# Autodesk Inventor assembly: NINA-W102 Module
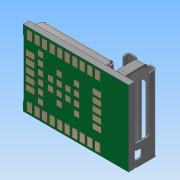
[picture p0: Inventor's stored thumbnail of the model, 180x180]
Saved by Autodesk Inventor 2016 (Build 200138000, 138)
## iProperties
Created: 2019-08-17
Part Number: NINA-W102 Module
Document SubType Name: Assembly
Designer: Orest
Catalog Web Link: https://www.u-blox.com/en/product/nina-w10-series; https://www.u-blox.com/sites/default/files/NINA-W10_DataSheet_%28UBX-17065507%29.pdf
Author: Orest
## Documents named in this file (4)
- E:\_Project TANK\Purchased\Arduino\Arduino NANO\Arduino NANO Every\NINA-W102\NINA-W102 Module.iam
- E:\_Project TANK\Purchased\Arduino\Arduino NANO\Arduino NANO Every\NINA-W102\NINA-W102 Antenna.ipt
- E:\_Project TANK\Purchased\Arduino\Arduino NANO\Arduino NANO Every\NINA-W102\NINA-W102 Body.ipt
- E:\_Project TANK\Purchased\Arduino\Arduino NANO\Arduino NANO Every\NINA-W102\NINA-W102 Cover.ipt
## Components (3 placed, 3 different names)
1. NINA-W102 Body:1 — Flush:1, Flush:2, Flush:3, Mate:1, Flush:5, Mate:2, Flush:7
2. NINA-W102 Antenna:1 — Mate:2, Flush:6, Flush:7
3. NINA-W102 Cover:1 — Mate:1, Flush:4, Flush:5
## Relationships (9: Flush 7, Mate 2)
- Flush:1: NINA-W102 Body:1
- Flush:2: NINA-W102 Body:1
- Flush:3: NINA-W102 Body:1
- Mate:1: NINA-W102 Body:1 ↔ NINA-W102 Cover:1
- Flush:4: NINA-W102 Cover:1
- Flush:5 (-0.4 mm): NINA-W102 Body:1 ↔ NINA-W102 Cover:1
- Mate:2: NINA-W102 Body:1 ↔ NINA-W102 Antenna:1
- Flush:6: NINA-W102 Antenna:1
- Flush:7: NINA-W102 Body:1 ↔ NINA-W102 Antenna:1
